# Autodesk Inventor assembly: SFX-100_ASSY
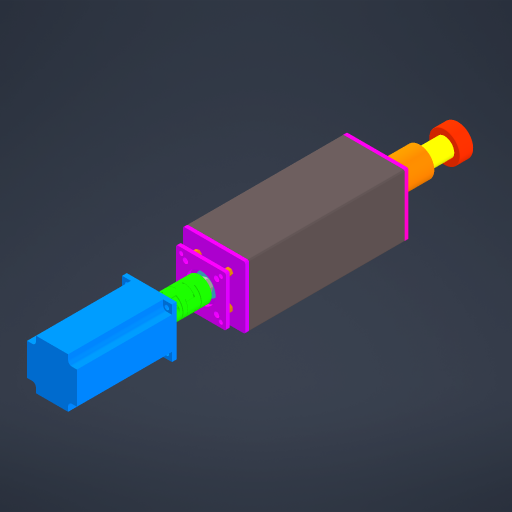
[picture p0: Inventor's stored thumbnail of the model, 512x512]
Saved by Autodesk Inventor 2023 (Build 270158000, 158)
## iProperties
Created: 2025-09-03
Part Number: SFX-100_ASSY
Document SubType Name: Assembly
Designer: k
Author: k
## Documents named in this file (16)
- C:\Users\k\Documents\SFX-100 100100W 제작\SFX-100_ASSY.iam
- C:\Users\k\Documents\SFX-100 100100W 제작\100100W-PROFILE.ipt
- C:\Users\k\Documents\SFX-100 100100W 제작\80AST-A1C02430.ipt
- C:\Users\k\Documents\SFX-100 100100W 제작\FK12.ipt
- C:\Users\k\Documents\SFX-100 100100W 제작\LMEK30UU.ipt
- C:\Users\k\Documents\SFX-100 100100W 제작\PL_BOTTOM.ipt
- C:\Users\k\Documents\SFX-100 100100W 제작\PL_TOP.ipt
- C:\Users\k\Documents\SFX-100 100100W 제작\hollow linear shaft.ipt
- C:\Users\k\Documents\SFX-100 100100W 제작\SFU1605_250mm.ipt
- C:\Users\k\Documents\Inventor\Content Center Files\R2023\ko-KR\DIN 934\DIN 934 - M12 x 1.75.ipt
- C:\Users\k\Documents\SFX-100 100100W 제작\Kupplung BG.iam
- C:\Users\k\Documents\SFX-100 100100W 제작\PL_TOP_1.ipt
- C:\Users\k\Documents\SFX-100 100100W 제작\BOLT_STUD_M8_15.ipt
- C:\Users\k\Documents\SFX-100 100100W 제작\SLIDER_80.ipt
- C:\Users\k\Documents\SFX-100 100100W 제작\BALL_NUT.ipt
- C:\Users\k\Documents\SFX-100 100100W 제작\FOOT.ipt
## Components (18 placed, 15 different names)
1. 100100W-PROFILE:1 — 메이트:2, 메이트:3, 메이트:6, 메이트:7, 메이트:8, 메이트:12, 메이트:20, 각도:1
2. 80AST-A1C02430:1 — 메이트:19, 메이트:21
3. FK12:1 — 메이트:4, 메이트:5, 메이트:9, 메이트:14, 메이트:15, 메이트:17
4. LMEK30UU:1 — 메이트:37, 메이트:38, 메이트:39, 메이트:40
5. PL_BOTTOM:1 — 메이트:2, 메이트:7, 메이트:12, 메이트:37, 메이트:38, 메이트:39
6. PL_TOP_2:1 — 메이트:3, 메이트:4, 메이트:5, 메이트:6, 메이트:8, 메이트:9, 메이트:23, 메이트:24, 메이트:25, 메이트:26, 메이트:27, 메이트:28, 메이트:29, 메이트:30
7. hollow linear shaft:1 — 메이트:32, 메이트:33, 메이트:40, 메이트:41, 메이트:42
8. SFU1605_250mm:1 — 메이트:14, 메이트:15, 메이트:16, 메이트:18, 메이트:22
9. DIN 934 - 다음으로 대치(됨): DIN EN 24032/28673/28674 M12:1 — 메이트:16, 메이트:17
10. 3 Jaw Coupling D40_10x19:1 [sub-assembly] — 메이트:18, 메이트:19, 메이트:22
11. PL_TOP_1:1 — 메이트:20, 메이트:21, 메이트:31
12. BOLT_STUD_M8_15:1 — 메이트:23, 메이트:24
13. BOLT_STUD_M8_15:2 — 메이트:25, 메이트:30
14. BOLT_STUD_M8_15:3 — 메이트:27, 메이트:29
15. BOLT_STUD_M8_15:4 — 메이트:26, 메이트:28, 메이트:31
16. SLIDER_80:1 — 메이트:32, 메이트:33, 메이트:34, 메이트:35, 각도:1, 메이트:36
17. BALL_NUT:1 — 메이트:34, 메이트:35, 메이트:36
18. FOOT:1 — 메이트:41, 메이트:42
## Relationships (39: Mate 38, Angle 1)
- 메이트:2 [Mate]: 100100W-PROFILE:1 ↔ PL_BOTTOM:1
- 메이트:3 [Mate]: 100100W-PROFILE:1 ↔ PL_TOP_2:1
- 메이트:4 [Mate]: FK12:1 ↔ PL_TOP_2:1
- 메이트:5 [Mate]: FK12:1 ↔ PL_TOP_2:1
- 메이트:6 [Mate]: 100100W-PROFILE:1 ↔ PL_TOP_2:1
- 메이트:7 [Mate]: 100100W-PROFILE:1 ↔ PL_BOTTOM:1
- 메이트:8 [Mate]: 100100W-PROFILE:1 ↔ PL_TOP_2:1
- 메이트:9 [Mate]: FK12:1 ↔ PL_TOP_2:1
- 메이트:12 [Mate]: 100100W-PROFILE:1 ↔ PL_BOTTOM:1
- 메이트:14 [Mate]: FK12:1 ↔ SFU1605_250mm:1
- 메이트:15 [Mate]: FK12:1 ↔ SFU1605_250mm:1
- 메이트:16 [Mate]: SFU1605_250mm:1 ↔ DIN 934 - 다음으로 대치(됨): DIN EN 24032/28673/28674 M12:1
- 메이트:17 [Mate]: FK12:1 ↔ DIN 934 - 다음으로 대치(됨): DIN EN 24032/28673/28674 M12:1
- 메이트:18 [Mate]: SFU1605_250mm:1 ↔ 3 Jaw Coupling D40_10x19:1
- 메이트:19 [Mate]: 80AST-A1C02430:1 ↔ 3 Jaw Coupling D40_10x19:1
- 메이트:20 [Mate]: 100100W-PROFILE:1 ↔ PL_TOP_1:1
- 메이트:21 [Mate]: 80AST-A1C02430:1 ↔ PL_TOP_1:1
- 메이트:22 [Mate]: SFU1605_250mm:1 ↔ 3 Jaw Coupling D40_10x19:1
- 메이트:23 [Mate]: PL_TOP_2:1 ↔ BOLT_STUD_M8_15:1
- 메이트:24 [Mate]: PL_TOP_2:1 ↔ BOLT_STUD_M8_15:1
- 메이트:25 [Mate]: PL_TOP_2:1 ↔ BOLT_STUD_M8_15:2
- 메이트:26 [Mate]: PL_TOP_2:1 ↔ BOLT_STUD_M8_15:4
- 메이트:27 [Mate]: PL_TOP_2:1 ↔ BOLT_STUD_M8_15:3
- 메이트:28 [Mate]: PL_TOP_2:1 ↔ BOLT_STUD_M8_15:4
- 메이트:29 [Mate]: PL_TOP_2:1 ↔ BOLT_STUD_M8_15:3
- 메이트:30 [Mate]: PL_TOP_2:1 ↔ BOLT_STUD_M8_15:2
- 메이트:31 [Mate]: PL_TOP_1:1 ↔ BOLT_STUD_M8_15:4
- 메이트:32 [Mate]: hollow linear shaft:1 ↔ SLIDER_80:1
- 메이트:33 [Mate]: hollow linear shaft:1 ↔ SLIDER_80:1
- 메이트:34 [Mate]: SLIDER_80:1 ↔ BALL_NUT:1
- 메이트:35 [Mate]: SLIDER_80:1 ↔ BALL_NUT:1
- 각도:1 [Angle] (0 deg): 100100W-PROFILE:1 ↔ SLIDER_80:1
- 메이트:36 [Mate]: SLIDER_80:1 ↔ BALL_NUT:1
- 메이트:37 [Mate]: LMEK30UU:1 ↔ PL_BOTTOM:1
- 메이트:38 [Mate]: LMEK30UU:1 ↔ PL_BOTTOM:1
- 메이트:39 [Mate]: LMEK30UU:1 ↔ PL_BOTTOM:1
- 메이트:40 [Mate]: LMEK30UU:1 ↔ hollow linear shaft:1
- 메이트:41 [Mate]: hollow linear shaft:1 ↔ FOOT:1
- 메이트:42 [Mate]: hollow linear shaft:1 ↔ FOOT:1
